# Autodesk Inventor assembly: VP_Input_to_2X_Ring_Gears_to_90_Degree_to_VP_Output_MIR
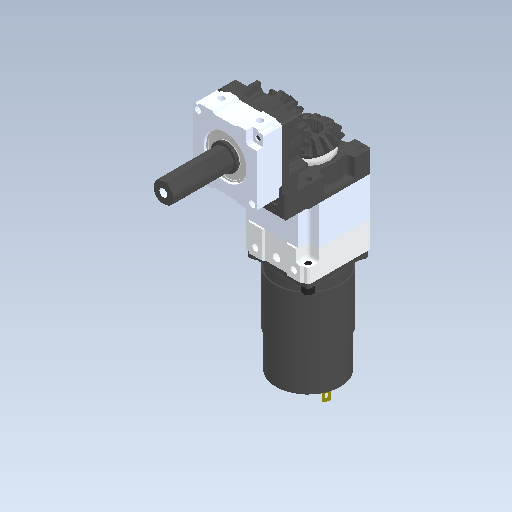
[picture p0: Inventor's stored thumbnail of the model, 512x512]
Saved by Autodesk Inventor 2020 (Build 240168000, 168)
## iProperties
Created: 2018-09-07
Part Number: VP_Input_to_2X_Ring_Gears_to_90_Degree_to_VP_Output_MIR
Description: STEP AP214
Document SubType Name: Assembly
Designer: Collin
Title: VP Input to 2X Ring Gears to 90 Degree to VP Output.STEP
Revision Number: ANY
Sending System: SolidWorks 2017
Preprocessor: SwSTEP 2.0
## Documents named in this file (14)
- D:\My Docs\Robotics\Robot Stuff\STEP Files\VPs\2 Stage VP 90Deg\VP_Input_to_2X_Ring_Gears_to_90_Degree_to_VP_Output_MIR.iam
- D:\My Docs\Robotics\Robot Stuff\STEP Files\VPs\2 Stage VP 90Deg\217-6293-000 Rev1_MIR.iam
- D:\My Docs\Robotics\Robot Stuff\STEP Files\VPs\2 Stage VP 90Deg\VersaPlanetary Input Blocks_VP Input Block_MIR.iam
- D:\My Docs\Robotics\Robot Stuff\STEP Files\VPs\2 Stage VP 90Deg\VersaPlanetary Output Blocks_VP Output Block_MIR.iam
- D:\My Docs\Robotics\Robot Stuff\STEP Files\VPs\2 Stage VP 90Deg\VersaPlanetary Output Shafts_0.500_ Hex (217-2615-003)_MIR.iam
- D:\My Docs\Robotics\Robot Stuff\STEP Files\VPs\2 Stage VP 90Deg\VersaPlanetary Ring Gears_VP Ring Gear_MIR.iam
- D:\My Docs\Robotics\Robot Stuff\STEP Files\VPs\2 Stage VP 90Deg\217-2816-001 Rev1_MIR.ipt
- D:\My Docs\Robotics\Robot Stuff\STEP Files\VPs\2 Stage VP 90Deg\VersaPlanetary Gear Sets_10_1 (217-2820)_MIR.iam
- D:\My Docs\Robotics\Robot Stuff\STEP Files\VPs\2 Stage VP 90Deg\217-2820-000 Rev2_Public_MIR.iam
- D:\My Docs\Robotics\Robot Stuff\STEP Files\VPs\2 Stage VP 90Deg\#8-32 SHCS, Grade 8 Steel Rev2_SSA0832-2250ZB_MIR.ipt
- D:\My Docs\Robotics\Robot Stuff\STEP Files\VPs\2 Stage VP 90Deg\#8-32 SHCS, Grade 8 Steel Rev2_SSA0832-0875ZB_MIR.ipt
- D:\My Docs\Robotics\Robot Stuff\STEP Files\VPs\2 Stage VP with 775pro\775pro_217-4347_MIR.ipt
- D:\My Docs\Robotics\Robot Stuff\STEP Files\VPs\2 Stage VP with 775pro\217-4649-002 Rev1_SSA0832-0500ZC_MIR.ipt
- D:\My Docs\Robotics\Robot Stuff\STEP Files\VPs\2 Stage VP with 775pro\217-2822-003 Rev4_MIR.ipt
## Components (16 placed, 13 different names)
1. 217-6293-000 Rev1_MIR:1 [sub-assembly]
2. VersaPlanetary Input Blocks_VP Input Block_MIR:1 [sub-assembly] — Mate:8, Angle:2, Mate:7
3. VersaPlanetary Output Blocks_VP Output Block_MIR:1 [sub-assembly]
4. VersaPlanetary Output Shafts_0.500_ Hex (217-2615-003)_MIR:1 [sub-assembly]
5. VersaPlanetary Ring Gears_VP Ring Gear_MIR:1 [sub-assembly]
6. 217-2816-001 Rev1_MIR:1
7. VersaPlanetary Gear Sets_10_1 (217-2820)_MIR:1 [sub-assembly]
8. 217-2820-000 Rev2_Public_MIR:1 [sub-assembly]
9. #8-32 SHCS, Grade 8 Steel Rev2_SSA0832-2250ZB_MIR:1
10. #8-32 SHCS, Grade 8 Steel Rev2_SSA0832-0875ZB_MIR:1
11. #8-32 SHCS, Grade 8 Steel Rev2_SSA0832-0875ZB_MIR:2
12. #8-32 SHCS, Grade 8 Steel Rev2_SSA0832-2250ZB_MIR:2
13. 775pro_217-4347_MIR:1 — Mate:2, Angle:1, Mate:1
14. 217-4649-002 Rev1_SSA0832-0500ZC_MIR:1 — Mate:8, Mate:5, Mate:4
15. 217-4649-002 Rev1_SSA0832-0500ZC_MIR:2 — Mate:6, Mate:3
16. 217-2822-003 Rev4_MIR:1 — Angle:2, Mate:7, Mate:6, Mate:5, Mate:4, Mate:3, Mate:2, Angle:1, Mate:1
## Relationships (10: Mate 8, Angle 2)
- Mate:8: VersaPlanetary Input Blocks_VP Input Block_MIR:1 ↔ 217-4649-002 Rev1_SSA0832-0500ZC_MIR:1
- Angle:2 (0 deg): VersaPlanetary Input Blocks_VP Input Block_MIR:1 ↔ 217-2822-003 Rev4_MIR:1
- Mate:7: VersaPlanetary Input Blocks_VP Input Block_MIR:1 ↔ 217-2822-003 Rev4_MIR:1
- Mate:6: 217-4649-002 Rev1_SSA0832-0500ZC_MIR:2 ↔ 217-2822-003 Rev4_MIR:1
- Mate:5: 217-4649-002 Rev1_SSA0832-0500ZC_MIR:1 ↔ 217-2822-003 Rev4_MIR:1
- Mate:4: 217-4649-002 Rev1_SSA0832-0500ZC_MIR:1 ↔ 217-2822-003 Rev4_MIR:1
- Mate:3: 217-4649-002 Rev1_SSA0832-0500ZC_MIR:2 ↔ 217-2822-003 Rev4_MIR:1
- Mate:2: 775pro_217-4347_MIR:1 ↔ 217-2822-003 Rev4_MIR:1
- Angle:1 (0 deg): 775pro_217-4347_MIR:1 ↔ 217-2822-003 Rev4_MIR:1
- Mate:1: 775pro_217-4347_MIR:1 ↔ 217-2822-003 Rev4_MIR:1
